# Autodesk Inventor assembly: robot2
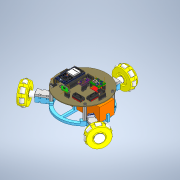
[picture p0: Inventor's stored thumbnail of the model, 180x180]
Saved by Autodesk Inventor 2020.2 (Build 242310000, 310)
## iProperties
Created: 2020-03-23
Part Number: robot2
Document SubType Name: Assembly
Designer: Tarsoly
Author: Tarsoly
## Documents named in this file (8)
- D:\Users\Tarsoly\Dokumentumok\BME\8. Félév\Önlab\3d\robot2.iam
- D:\Users\Tarsoly\Dokumentumok\BME\8. Félév\Önlab\3d\bottom2.ipt
- D:\Users\Tarsoly\Dokumentumok\BME\8. Félév\Önlab\3d\akksi.ipt
- D:\Users\Tarsoly\Dokumentumok\BME\8. Félév\Önlab\3d\tavtarto_30mm.ipt
- D:\Users\Tarsoly\Dokumentumok\BME\8. Félév\Önlab\3d\electronics.iam
- D:\Users\Tarsoly\Dokumentumok\BME\8. Félév\Önlab\3d\power_train.iam
- D:\Users\Tarsoly\Documents\Inventor\Content Center Files\R2020\en-US\ISO 4762(2)\ISO 4762 - M3 x 6ISO.ipt
- D:\Users\Tarsoly\Dokumentumok\BME\8. Félév\Önlab\3d\motor_top.ipt
## Components (21 placed, 7 different names)
1. bottom2:1 — Mate:1, Flush:1, Mate:2, Mate:3, Mate:4, Angle:1, Mate:10, Mate:11, Mate:12, Mate:13, Angle:2, Angle:3, Angle:4, Angle:5, Mate:14, Mate:15, Mate:16, Angle:6, Mate:23, Mate:24, Mate:25, Mate:26, Flush:2, Flush:3, Mate:39, Mate:40, Mate:41, Mate:42, Mate:43
2. akksi:1 — Mate:14, Mate:15, Mate:16
3. electronics:1 [sub-assembly] — Mate:17, Mate:18, Angle:6, Mate:19, Mate:20, Mate:21, Mate:28, Mate:32, Mate:33, Mate:34, Mate:36, Mate:37, Mate:38
4. tavtarto_30mm:1 — Mate:11, Angle:4, Mate:36
5. tavtarto_30mm:2 — Mate:13, Angle:3, Mate:22, Mate:38
6. tavtarto_30mm:3 — Mate:12, Angle:2, Mate:17, Mate:18
7. tavtarto_30mm:4 — Mate:10, Angle:5, Mate:37, Mate:39
8. ISO 4762 M3 x 6:1 — Mate:20, Mate:32
9. ISO 4762 M3 x 6:2 — Mate:19, Mate:33
10. ISO 4762 M3 x 6:5 — Mate:22, Mate:34
11. ISO 4762 M3 x 6:6 — Mate:21, Mate:28
12. ISO 4762 M3 x 6:3 — Mate:23, Mate:41
13. ISO 4762 M3 x 6:4 — Mate:25, Mate:40
14. ISO 4762 M3 x 6:7 — Mate:24, Mate:42
15. ISO 4762 M3 x 6:8 — Mate:26, Mate:43
16. power_train:1 [sub-assembly] — Mate:2, Mate:3, Mate:4
17. power_train:2 [sub-assembly] — Tangent:1, Mate:35
18. power_train:3 [sub-assembly]
19. motor_top:1 — Mate:35, Flush:2, Flush:3
20. motor_top:2
21. motor_top:3
## Component patterns: powertrains (3 elements), (3 elements, first: motor_top:1)
## Relationships (45: Mate 35, Angle 6, Flush 3, Tangent 1)
- Mate:1 (-2.5 mm): bottom2:1
- Flush:1 (-2.5 mm): bottom2:1
- Mate:2: bottom2:1 ↔ power_train:1
- Mate:3: bottom2:1 ↔ power_train:1
- Mate:4: bottom2:1 ↔ power_train:1
- Angle:1 (0 deg): bottom2:1
- Tangent:1: power_train:2
- Mate:5
- Mate:10: bottom2:1 ↔ tavtarto_30mm:4
- Mate:11: bottom2:1 ↔ tavtarto_30mm:1
- Mate:12: bottom2:1 ↔ tavtarto_30mm:3
- Mate:13: bottom2:1 ↔ tavtarto_30mm:2
- Angle:2 (0 deg): bottom2:1 ↔ tavtarto_30mm:3
- Angle:3 (0 deg): bottom2:1 ↔ tavtarto_30mm:2
- Angle:4 (0 deg): bottom2:1 ↔ tavtarto_30mm:1
- Angle:5 (0 deg): bottom2:1 ↔ tavtarto_30mm:4
- Mate:14: bottom2:1 ↔ akksi:1
- Mate:15 (0.2 mm): bottom2:1 ↔ akksi:1
- Mate:16 (0.2 mm): bottom2:1 ↔ akksi:1
- Mate:17: electronics:1 ↔ tavtarto_30mm:3
- Mate:18: electronics:1 ↔ tavtarto_30mm:3
- Angle:6 (0 deg): bottom2:1 ↔ electronics:1
- Mate:19: electronics:1 ↔ ISO 4762 M3 x 6:2
- Mate:20: electronics:1 ↔ ISO 4762 M3 x 6:1
- Mate:21: electronics:1 ↔ ISO 4762 M3 x 6:6
- Mate:22: tavtarto_30mm:2 ↔ ISO 4762 M3 x 6:5
- Mate:23: bottom2:1 ↔ ISO 4762 M3 x 6:3
- Mate:24: bottom2:1 ↔ ISO 4762 M3 x 6:7
- Mate:25: bottom2:1 ↔ ISO 4762 M3 x 6:4
- Mate:26: bottom2:1 ↔ ISO 4762 M3 x 6:8
- Mate:28: electronics:1 ↔ ISO 4762 M3 x 6:6
- Mate:32: electronics:1 ↔ ISO 4762 M3 x 6:1
- Mate:33: electronics:1 ↔ ISO 4762 M3 x 6:2
- Mate:34: electronics:1 ↔ ISO 4762 M3 x 6:5
- Mate:35: power_train:2 ↔ motor_top:1
- Flush:2: bottom2:1 ↔ motor_top:1
- Flush:3: bottom2:1 ↔ motor_top:1
- Mate:36: electronics:1 ↔ tavtarto_30mm:1
- Mate:37: electronics:1 ↔ tavtarto_30mm:4
- Mate:38: electronics:1 ↔ tavtarto_30mm:2
- Mate:39: bottom2:1 ↔ tavtarto_30mm:4
- Mate:40: bottom2:1 ↔ ISO 4762 M3 x 6:4
- Mate:41: bottom2:1 ↔ ISO 4762 M3 x 6:3
- Mate:42: bottom2:1 ↔ ISO 4762 M3 x 6:7
- Mate:43: bottom2:1 ↔ ISO 4762 M3 x 6:8
